# Autodesk Inventor assembly: gearbox
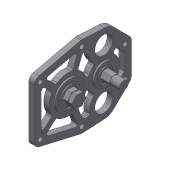
[picture p0: Inventor's stored thumbnail of the model, 180x180]
Saved by Autodesk Inventor 2013 SP1 (Build 170176100, 176)
## iProperties
Created: 2013-11-05
Part Number: gearbox
Document SubType Name: Assembly
Designer: robotics
Author: robotics
## Documents named in this file (6)
- C:\Users\robotics\Documents\GitHub\2014-Preseason-Single-Speed-Gearbox\custom\gearbox.iam
- C:\Users\robotics\Documents\GitHub\2014-Preseason-Single-Speed-Gearbox\custom\BackPlate.ipt
- C:\Users\robotics\Documents\GitHub\2014-Preseason-Single-Speed-Gearbox\custom\LongShaft.ipt
- C:\Users\robotics\Documents\GitHub\2014-Preseason-Single-Speed-Gearbox\custom\RoundBearing-1-2-inch.ipt
- C:\Users\robotics\Documents\GitHub\2014-Preseason-Single-Speed-Gearbox\custom\RoundBearing-3-8-inch.ipt
- C:\Users\robotics\Documents\GitHub\2014-Preseason-Single-Speed-Gearbox\custom\ShortShaft.ipt
## Components (5 placed, 5 different names)
1. BackPlate:1 — Mate:1, Mate:2, Mate:5, Mate:6
2. LongShaft:1 — Mate:3, Mate:4
3. RoundBearing-1-2-inch:1 — Mate:1, Mate:2, Mate:3, Mate:4
4. RoundBearing-3-8-inch:1 — Mate:5, Mate:6, Mate:7, Mate:8
5. ShortShaft:1 — Mate:7, Mate:8
## Relationships (8: Mate 8)
- Mate:1: BackPlate:1 ↔ RoundBearing-1-2-inch:1
- Mate:2: BackPlate:1 ↔ RoundBearing-1-2-inch:1
- Mate:3: LongShaft:1 ↔ RoundBearing-1-2-inch:1
- Mate:4: LongShaft:1 ↔ RoundBearing-1-2-inch:1
- Mate:5: BackPlate:1 ↔ RoundBearing-3-8-inch:1
- Mate:6: BackPlate:1 ↔ RoundBearing-3-8-inch:1
- Mate:7: RoundBearing-3-8-inch:1 ↔ ShortShaft:1
- Mate:8: RoundBearing-3-8-inch:1 ↔ ShortShaft:1
